# Autodesk Inventor assembly: Chasis
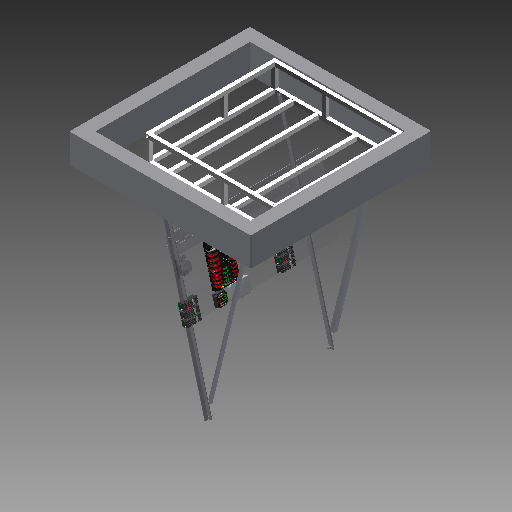
[picture p0: Inventor's stored thumbnail of the model, 512x512]
Saved by Autodesk Inventor 2019.4 (Build 234330000, 330)
## iProperties
has-driver: False
num-sensors: 0
robot-weight-kg: 226.0
robot-prefer-metric: False
robot-driveTrainType: 3
has-driver: True
driver-type: 1
motor-type: 0
driver-port1: 1
driver-port2: -1
driver-isCan: False
driver-lowerLimit: 0.0
driver-upperLimit: 0.0
driver-inputGear: 0.0
driver-outputGear: 0.0
driver-hasBrake: False
has-wheel: True
wheel-type: 3
wheel-isDriveWheel: True
wheel-frictionLevel: 1
has-pneumatic: False
has-elevator: False
driver-port1: 0
Created: 2019-01-05
Part Number: Chasis
Document SubType Name: Assembly
Designer: Jacob's Laptop
Mass: 6918.42 g
Surface Area: 25184.8 cm^2
Volume: 3653.81 cm^3
Density: 1.89348 g/cm^3
Author: Jacob's Laptop
## Documents named in this file (21)
- D:\FIRST FRC\Synthesis Robots\Epsilon\Chasis\Chasis.iam
- D:\FIRST FRC\Synthesis Robots\Epsilon\Chasis\Chasis Long Length.ipt
- D:\FIRST FRC\Synthesis Robots\Epsilon\Chasis\Chasis Short Length.ipt
- D:\FIRST FRC\Synthesis Robots\Epsilon\Chasis\Chasis Hieght.ipt
- D:\FIRST FRC\Synthesis Robots\Epsilon\Chasis\AluminumLchannelLeft.ipt.iam
- D:\FIRST FRC\Synthesis Robots\Epsilon\Chasis\AluminumChannelRight.iam
- D:\FIRST FRC\Synthesis Robots\Epsilon\Chasis\Hinge\Piano hingehinge - Copy.ipt
- D:\FIRST FRC\Synthesis Robots\Epsilon\Chasis\Hinge\Piano hingehinge pin - Copy.ipt
- D:\FIRST FRC\Synthesis Robots\Epsilon\Swerve drive parts\10-24 Hex Washer Rolling x 3-4_93882A213.ipt
- D:\FIRST FRC\Synthesis Robots\Epsilon\Swerve drive parts\10-32 Nylock Nut 1_90631A411.ipt
- D:\FIRST FRC\Synthesis Robots\Epsilon\Chasis\am-1149 0.25'' Flat Washer, Stainless Steel REV2.ipt
- D:\FIRST FRC\Synthesis Robots\Epsilon\Chasis\Plexi Glass.ipt
- D:\FIRST FRC\Synthesis Robots\Epsilon\Chasis\OM5P-AN.ipt
- D:\FIRST FRC\Synthesis Robots\Epsilon\Chasis\Power_Distribution_Panel_217-4244 (1).ipt
- D:\FIRST FRC\Synthesis Robots\Epsilon\Chasis\Voltage_Regulator_Module_217-4245.ipt
- D:\FIRST FRC\Synthesis Robots\Epsilon\Chasis\Talons\Talon_SRX_217-8080_No_Wires.iam
- D:\FIRST FRC\Synthesis Robots\Epsilon\Chasis\am-0282 120a Circuit Breaker.ipt
- D:\FIRST FRC\Synthesis Robots\Epsilon\Chasis\AluminumChannelRight Copy.iam
- D:\FIRST FRC\Synthesis Robots\Epsilon\Chasis\AluminumLchannelLeft. Copyipt.iam
- D:\FIRST FRC\Synthesis Robots\Epsilon\Chasis\Bumpers.ipt
- AluminumLchannelLeft.ipt
## Components (47 placed, 19 different names)
1. Chasis Long Length:1 — Mate:1, Flush:1, Flush:2, Mate:2, Flush:3, Flush:4, Mate:3, Flush:5, Flush:6, Mate:6, Flush:12
2. Chasis Long Length:2 — Mate:4, Flush:7, Flush:8, Mate:5, Flush:9, Mate:7, Flush:13, Flush:14, Mate:79
3. Chasis Short Length:1 — Mate:2, Flush:3, Flush:4
4. Chasis Short Length:2 — Mate:3, Flush:5, Flush:6, Mate:4, Flush:7, Flush:8, Flush:10, Flush:11, Flush:24, Mate:80
5. Chasis Hieght:1 — Mate:1, Flush:1, Flush:2, Mate:11, Flush:21, Flush:22, Mate:13, Mate:17
6. Chasis Hieght:2 — Mate:6, Flush:11, Flush:12
7. Chasis Hieght:3 — Mate:5, Flush:9, Flush:10, Mate:15, Angle:1
8. Chasis Hieght:4 — Mate:7, Flush:13, Flush:14, Mate:19
9. Chasis Long Length:3 — Mate:11, Flush:21, Flush:22, Mate:16, Flush:25, Mate:29, Tangent:1, Mate:30, Mate:75, Mate:76
10. Chasis Long Length:4 — Mate:14, Mate:21, Flush:27, Mate:22, Flush:28, Mate:23, Flush:29, Mate:24, Flush:30, Mate:32, Mate:33, Mate:43, Mate:77, Mate:78, Flush:43
11. Chasis Short Length:3 — Mate:18, Flush:26, Mate:27
12. Chasis Short Length:4 — Mate:12, Flush:23, Mate:28
13. Chasis Hieght:5 — Mate:18, Flush:26, Mate:19
14. Chasis Hieght:6 — Mate:16, Flush:25, Mate:17
15. Chasis Hieght:7 — Mate:12, Flush:23, Mate:13
16. Chasis Hieght:8 — Mate:14, Flush:24, Mate:15
17. Chasis Short Length:5 — Mate:21, Flush:27, Mate:25, Mate:27
18. Chasis Short Length:6 — Mate:22, Flush:28, Mate:25
19. Chasis Short Length:7 — Mate:23, Flush:29, Mate:26
20. Chasis Short Length:8 — Mate:24, Flush:30, Mate:26, Mate:28
21. AluminumLchannelLeft.ipt:1 [sub-assembly] — Mate:29, Tangent:1, Mate:30, Flush:31, Flush:34
22. AluminumChannelRight:1 [sub-assembly] — Mate:32, Flush:31, Mate:33, Angle:1, Tangent:3, Mate:58
23. Piano hingehinge - Copy:1 — Flush:34, Mate:43, Mate:46, Tangent:4, Mate:48, Mate:52, Tangent:5, Tangent:6, Mate:54, Tangent:7, Tangent:10, Tangent:13
24. Piano hingehinge - Copy:2 — Mate:61, Flush:35
25. Piano hingehinge pin - Copy:1
26. 10-24 Hex Washer Rolling x 3-4_93882A213:2 — Mate:46, Tangent:3, Tangent:4, Mate:47, Mate:50, Mate:56
27. 10-32 Nylock Nut 1_90631A411:1 — Mate:55
28. 10-32 Nylock Nut 1_90631A411:2 — Mate:50
29. am-1149 0.25'' Flat Washer, Stainless Steel REV2:1 — Mate:47, Mate:48, Mate:57
30. am-1149 0.25'' Flat Washer, Stainless Steel REV2:2 — Mate:53, Mate:54, Mate:60
31. 10-24 Hex Washer Rolling x 3-4_93882A213:3 — Mate:52, Tangent:5, Tangent:6, Mate:53, Mate:55, Mate:59
32. am-1149 0.25'' Flat Washer, Stainless Steel REV2:3 — Mate:56, Mate:57, Mate:58
33. am-1149 0.25'' Flat Washer, Stainless Steel REV2:4 — Mate:59, Mate:60
34. Plexi Glass:1 — Mate:61, Flush:35, Tangent:7, Mate:62, Tangent:8, Tangent:9, Mate:63, Mate:64, Mate:65, Mate:66, Mate:67, Mate:68, Mate:69, Mate:70, Mate:71, Mate:72, Mate:73, Mate:74
35. OM5P-AN:1 — Mate:62, Tangent:8, Tangent:9
36. Power_Distribution_Panel_217-4244 (1):1 — Mate:63, Tangent:10
37. Voltage_Regulator_Module_217-4245:1 — Mate:64, Mate:70
38. Talon_SRX_217-8080_No_Wires:1 [sub-assembly] — Mate:66, Flush:37, Tangent:12, Mate:68
39. Talon_SRX_217-8080_No_Wires:2 [sub-assembly] — Mate:65, Flush:36, Tangent:11, Tangent:12
40. Talon_SRX_217-8080_No_Wires:3 [sub-assembly] — Mate:67, Flush:36, Flush:37, Tangent:11
41. am-0282 120a Circuit Breaker:1 — Mate:69, Tangent:13
42. Talon_SRX_217-8080_No_Wires:4 [sub-assembly] — Flush:40, Flush:41, Mate:71, Mate:74
43. Talon_SRX_217-8080_No_Wires:5 [sub-assembly] — Flush:41, Mate:72
44. Talon_SRX_217-8080_No_Wires:6 [sub-assembly] — Flush:40, Mate:73
45. AluminumChannelRight Copy:1 [sub-assembly] — Mate:75, Mate:76, Flush:42
46. AluminumLchannelLeft. Copyipt:1 [sub-assembly] — Mate:77, Flush:42, Mate:78
47. Bumpers:1 — Mate:79, Mate:80, Flush:43
## Relationships (125: Mate 69, Flush 41, Tangent 14, Angle 1)
- Mate:1: Chasis Long Length:1 ↔ Chasis Hieght:1
- Flush:1: Chasis Long Length:1 ↔ Chasis Hieght:1
- Flush:2: Chasis Long Length:1 ↔ Chasis Hieght:1
- Mate:2: Chasis Long Length:1 ↔ Chasis Short Length:1
- Flush:3: Chasis Long Length:1 ↔ Chasis Short Length:1
- Flush:4: Chasis Long Length:1 ↔ Chasis Short Length:1
- Mate:3: Chasis Long Length:1 ↔ Chasis Short Length:2
- Flush:5: Chasis Long Length:1 ↔ Chasis Short Length:2
- Flush:6: Chasis Long Length:1 ↔ Chasis Short Length:2
- Mate:4: Chasis Long Length:2 ↔ Chasis Short Length:2
- Flush:7: Chasis Long Length:2 ↔ Chasis Short Length:2
- Flush:8: Chasis Long Length:2 ↔ Chasis Short Length:2
- Mate:5: Chasis Long Length:2 ↔ Chasis Hieght:3
- Flush:9: Chasis Long Length:2 ↔ Chasis Hieght:3
- Flush:10: Chasis Short Length:2 ↔ Chasis Hieght:3
- Mate:6: Chasis Long Length:1 ↔ Chasis Hieght:2
- Flush:11: Chasis Short Length:2 ↔ Chasis Hieght:2
- Flush:12: Chasis Long Length:1 ↔ Chasis Hieght:2
- Mate:7: Chasis Long Length:2 ↔ Chasis Hieght:4
- Flush:13: Chasis Long Length:2 ↔ Chasis Hieght:4
- Flush:14: Chasis Long Length:2 ↔ Chasis Hieght:4
- [Mate]: Chasis Long Length:3 ↔ Chasis Short Length:3
- [Flush]: Chasis Long Length:3 ↔ Chasis Short Length:3
- [Flush]: Chasis Long Length:3 ↔ Chasis Short Length:3
- [Mate]: Chasis Long Length:3 ↔ Chasis Short Length:4
- [Flush]: Chasis Long Length:3 ↔ Chasis Short Length:4
- [Flush]: Chasis Long Length:3 ↔ Chasis Short Length:4
- [Mate]: Chasis Long Length:4 ↔ Chasis Short Length:4
- [Flush]: Chasis Long Length:4 ↔ Chasis Short Length:4
- [Flush]: Chasis Long Length:4 ↔ Chasis Short Length:4
- Mate:11: Chasis Hieght:1 ↔ Chasis Long Length:3
- Flush:21: Chasis Hieght:1 ↔ Chasis Long Length:3
- Flush:22: Chasis Hieght:1 ↔ Chasis Long Length:3
- Mate:12: Chasis Short Length:4 ↔ Chasis Hieght:7
- Flush:23: Chasis Short Length:4 ↔ Chasis Hieght:7
- Mate:13 (349.25 mm): Chasis Hieght:1 ↔ Chasis Hieght:7
- Mate:14: Chasis Long Length:4 ↔ Chasis Hieght:8
- Flush:24: Chasis Short Length:2 ↔ Chasis Hieght:8
- Mate:15 (349.25 mm): Chasis Hieght:3 ↔ Chasis Hieght:8
- Mate:16: Chasis Long Length:3 ↔ Chasis Hieght:6
- Flush:25: Chasis Long Length:3 ↔ Chasis Hieght:6
- Mate:17 (349.25 mm): Chasis Hieght:1 ↔ Chasis Hieght:6
- Mate:18: Chasis Short Length:3 ↔ Chasis Hieght:5
- Flush:26: Chasis Short Length:3 ↔ Chasis Hieght:5
- Mate:19 (349.25 mm): Chasis Hieght:4 ↔ Chasis Hieght:5
- Mate:21: Chasis Long Length:4 ↔ Chasis Short Length:5
- Flush:27: Chasis Long Length:4 ↔ Chasis Short Length:5
- Mate:22: Chasis Long Length:4 ↔ Chasis Short Length:6
- Flush:28: Chasis Long Length:4 ↔ Chasis Short Length:6
- Mate:23: Chasis Long Length:4 ↔ Chasis Short Length:7
- Flush:29: Chasis Long Length:4 ↔ Chasis Short Length:7
- Mate:24: Chasis Long Length:4 ↔ Chasis Short Length:8
- Flush:30: Chasis Long Length:4 ↔ Chasis Short Length:8
- Mate:25 (101.6 mm): Chasis Short Length:5 ↔ Chasis Short Length:6
- Mate:26 (101.6 mm): Chasis Short Length:7 ↔ Chasis Short Length:8
- Mate:27 (76.2 mm): Chasis Short Length:3 ↔ Chasis Short Length:5
- Mate:28 (76.2 mm): Chasis Short Length:4 ↔ Chasis Short Length:8
- Mate:29: Chasis Long Length:3 ↔ AluminumLchannelLeft.ipt:1
- Tangent:1 (38.1 mm): Chasis Long Length:3 ↔ AluminumLchannelLeft.ipt:1
- Mate:30: Chasis Long Length:3 ↔ AluminumLchannelLeft.ipt:1
- Mate:32: Chasis Long Length:4 ↔ AluminumChannelRight:1
- Flush:31: AluminumLchannelLeft.ipt:1 ↔ AluminumChannelRight:1
- Mate:33: Chasis Long Length:4 ↔ AluminumChannelRight:1
- Angle:1 (285 deg): Chasis Hieght:3 ↔ AluminumChannelRight:1
- [Mate]: Piano hingehinge - Copy:2 ↔ Piano hingehinge pin - Copy:1
- [Mate]: Piano hingehinge - Copy:1 ↔ Piano hingehinge pin - Copy:1
- [Mate]: Piano hingehinge - Copy:1 ↔ Piano hingehinge - Copy:2
- [Mate]: Piano hingehinge - Copy:2 ↔ Piano hingehinge pin - Copy:1
- Flush:34: AluminumLchannelLeft.ipt:1 ↔ Piano hingehinge - Copy:1
- Mate:43 (254 mm): Chasis Long Length:4 ↔ Piano hingehinge - Copy:1
- Mate:46: Piano hingehinge - Copy:1 ↔ 10-24 Hex Washer Rolling x 3-4_93882A213:2
- Tangent:3 (-15.24 mm): AluminumChannelRight:1 ↔ 10-24 Hex Washer Rolling x 3-4_93882A213:2
- Tangent:4 (6.35 mm): Piano hingehinge - Copy:1 ↔ 10-24 Hex Washer Rolling x 3-4_93882A213:2
- Mate:47: 10-24 Hex Washer Rolling x 3-4_93882A213:2 ↔ am-1149 0.25'' Flat Washer, Stainless Steel REV2:1
- Mate:48: Piano hingehinge - Copy:1 ↔ am-1149 0.25'' Flat Washer, Stainless Steel REV2:1
- Mate:50: 10-24 Hex Washer Rolling x 3-4_93882A213:2 ↔ 10-32 Nylock Nut 1_90631A411:2
- Mate:52: Piano hingehinge - Copy:1 ↔ 10-24 Hex Washer Rolling x 3-4_93882A213:3
- Tangent:5 (-12.7 mm): Piano hingehinge - Copy:1 ↔ 10-24 Hex Washer Rolling x 3-4_93882A213:3
- Tangent:6 (-12.7 mm): Piano hingehinge - Copy:1 ↔ 10-24 Hex Washer Rolling x 3-4_93882A213:3
- Mate:53: am-1149 0.25'' Flat Washer, Stainless Steel REV2:2 ↔ 10-24 Hex Washer Rolling x 3-4_93882A213:3
- Mate:54: Piano hingehinge - Copy:1 ↔ am-1149 0.25'' Flat Washer, Stainless Steel REV2:2
- Mate:55: 10-32 Nylock Nut 1_90631A411:1 ↔ 10-24 Hex Washer Rolling x 3-4_93882A213:3
- Mate:56: 10-24 Hex Washer Rolling x 3-4_93882A213:2 ↔ am-1149 0.25'' Flat Washer, Stainless Steel REV2:3
- Mate:57: am-1149 0.25'' Flat Washer, Stainless Steel REV2:1 ↔ am-1149 0.25'' Flat Washer, Stainless Steel REV2:3
- Mate:58: AluminumChannelRight:1 ↔ am-1149 0.25'' Flat Washer, Stainless Steel REV2:3
- Mate:59: 10-24 Hex Washer Rolling x 3-4_93882A213:3 ↔ am-1149 0.25'' Flat Washer, Stainless Steel REV2:4
- Mate:60: am-1149 0.25'' Flat Washer, Stainless Steel REV2:2 ↔ am-1149 0.25'' Flat Washer, Stainless Steel REV2:4
- Mate:61: Piano hingehinge - Copy:2 ↔ Plexi Glass:1
- Flush:35: Piano hingehinge - Copy:2 ↔ Plexi Glass:1
- Tangent:7: Piano hingehinge - Copy:1 ↔ Plexi Glass:1
- Mate:62: Plexi Glass:1 ↔ OM5P-AN:1
- Tangent:8 (6.35 mm): Plexi Glass:1 ↔ OM5P-AN:1
- Tangent:9 (6.35 mm): Plexi Glass:1 ↔ OM5P-AN:1
- Mate:63: Plexi Glass:1 ↔ Power_Distribution_Panel_217-4244 (1):1
- Tangent:10 (38.1 mm): Piano hingehinge - Copy:1 ↔ Power_Distribution_Panel_217-4244 (1):1
- Mate:64: Plexi Glass:1 ↔ Voltage_Regulator_Module_217-4245:1
- Mate:65: Plexi Glass:1 ↔ Talon_SRX_217-8080_No_Wires:2
- Mate:66: Plexi Glass:1 ↔ Talon_SRX_217-8080_No_Wires:1
- Mate:67: Plexi Glass:1 ↔ Talon_SRX_217-8080_No_Wires:3
- Flush:36: Talon_SRX_217-8080_No_Wires:2 ↔ Talon_SRX_217-8080_No_Wires:3
- Flush:37: Talon_SRX_217-8080_No_Wires:1 ↔ Talon_SRX_217-8080_No_Wires:3
- Tangent:11 (6.35 mm): Talon_SRX_217-8080_No_Wires:2 ↔ Talon_SRX_217-8080_No_Wires:3
- Tangent:12 (6.35 mm): Talon_SRX_217-8080_No_Wires:1 ↔ Talon_SRX_217-8080_No_Wires:2
- Mate:68 (-6.35 mm): Plexi Glass:1 ↔ Talon_SRX_217-8080_No_Wires:1
- Mate:69: Plexi Glass:1 ↔ am-0282 120a Circuit Breaker:1
- Tangent:13 (44.45 mm): Piano hingehinge - Copy:1 ↔ am-0282 120a Circuit Breaker:1
- Mate:70 (-6.35 mm): Plexi Glass:1 ↔ Voltage_Regulator_Module_217-4245:1
- [Flush]: Talon_SRX_217-8080_No_Wires:5 ↔ Talon_SRX_217-8080_No_Wires:6
- [Flush]: Talon_SRX_217-8080_No_Wires:4 ↔ Talon_SRX_217-8080_No_Wires:6
- [Tangent] (6.35 mm): Talon_SRX_217-8080_No_Wires:5 ↔ Talon_SRX_217-8080_No_Wires:6
- [Tangent] (6.35 mm): Talon_SRX_217-8080_No_Wires:4 ↔ Talon_SRX_217-8080_No_Wires:5
- Flush:40: Talon_SRX_217-8080_No_Wires:4 ↔ Talon_SRX_217-8080_No_Wires:6
- Flush:41: Talon_SRX_217-8080_No_Wires:4 ↔ Talon_SRX_217-8080_No_Wires:5
- Mate:71: Plexi Glass:1 ↔ Talon_SRX_217-8080_No_Wires:4
- Mate:72: Plexi Glass:1 ↔ Talon_SRX_217-8080_No_Wires:5
- Mate:73: Plexi Glass:1 ↔ Talon_SRX_217-8080_No_Wires:6
- Mate:74 (-6.35 mm): Plexi Glass:1 ↔ Talon_SRX_217-8080_No_Wires:4
- Mate:75: Chasis Long Length:3 ↔ AluminumChannelRight Copy:1
- Mate:76: Chasis Long Length:3 ↔ AluminumChannelRight Copy:1
- Mate:77: Chasis Long Length:4 ↔ AluminumLchannelLeft. Copyipt:1
- Flush:42: AluminumChannelRight Copy:1 ↔ AluminumLchannelLeft. Copyipt:1
- Mate:78: Chasis Long Length:4 ↔ AluminumLchannelLeft. Copyipt:1
- Mate:79: Chasis Long Length:2 ↔ Bumpers:1
- Mate:80: Chasis Short Length:2 ↔ Bumpers:1
- Flush:43: Chasis Long Length:4 ↔ Bumpers:1
## Named parameters: d21_d3 = 0 mm, d22_d4 = 0 mm, d23_d5 = 0 mm, d24_d6 = 0 mm, d25_d7 = 0 mm, d26_d8 = 0 mm, d27_d9 = 0 mm, d28_d10 = 0 mm, d29_d11 = 0 mm, d803_d0 = 0 mm, d804_d2 = 0 mm, d805_d5 = 0 mm, d806_d6 = 0 mm, d886_d878 = 0 mm, d887_d879 = 0 mm, d888_d880 = 6.35 mm, d889_d881 = 6.35 mm
